# Autodesk Inventor assembly: Bar Cabinet Assembly
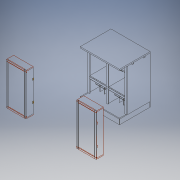
[picture p0: Inventor's stored thumbnail of the model, 180x180]
Saved by Autodesk Inventor 2016 (Build 200138000, 138)
## iProperties
Created: 2017-10-30
Part Number: Bar Cabinet Assembly
Document SubType Name: Assembly
Designer: mathaetaes
Author: mathaetaes
## Documents named in this file (4)
- E:\Projects\3D Printer\printer projects\My Designs\Bar Cabinet 2.20.2018\001 Bar Cabinet Full Assembly.iam
- E:\Projects\3D Printer\printer projects\My Designs\Bar Cabinet 2.20.2018\Door 2.iam
- E:\Projects\3D Printer\printer projects\My Designs\Bar Cabinet 2.20.2018\Bar Cabinet And Base.iam
- E:\Projects\3D Printer\printer projects\My Designs\Bar Cabinet 2.20.2018\Door.iam
## Components (3 placed, 3 different names)
1. Bar Cabinet And Base:1 [sub-assembly] — Mate:1, Mate:2
2. Door:1 [sub-assembly] — Flush:1, Mate:1
3. Door 2:1 [sub-assembly] — Flush:1, Mate:2
## Relationships (3: Mate 2, Flush 1)
- Flush:1: Door:1 ↔ Door 2:1
- Mate:1: Bar Cabinet And Base:1 ↔ Door:1
- Mate:2: Bar Cabinet And Base:1 ↔ Door 2:1
